# Autodesk Inventor assembly: Reactor Assembly
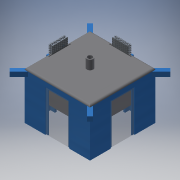
[picture p0: Inventor's stored thumbnail of the model, 180x180]
Saved by Autodesk Inventor 2017 (Build 210142000, 142)
## iProperties
Created: 2017-01-05
Part Number: Reactor Assembly
Document SubType Name: Assembly
Designer: jbui8
Author: jbui8
## Documents named in this file (5)
- C:\Users\jbui8\OneDrive\Documents\CAD Designs for Research and Work\PV Electrolyzer\Reactor Design\Reactor Parts\Assembly Parts\Reactor Assembly.iam
- C:\Users\jbui8\OneDrive\Documents\CAD Designs for Research and Work\PV Electrolyzer\Reactor Design\Reactor Parts\Assembly Parts\Reactor Main Body.ipt
- C:\Users\jbui8\OneDrive\Documents\CAD Designs for Research and Work\PV Electrolyzer\Reactor Design\Reactor Parts\Assembly Parts\Reactor Lid.ipt
- C:\Users\jbui8\OneDrive\Documents\CAD Designs for Research and Work\PV Electrolyzer\Reactor Design\Reactor Parts\Assembly Parts\Reactor Glass.ipt
- C:\Users\jbui8\OneDrive\Documents\CAD Designs for Research and Work\PV Electrolyzer\Reactor Design\Reactor Parts\Assembly Parts\Reactor Meshes.ipt
## Components (6 placed, 4 different names)
1. Reactor Main Body:1 — Mate:1, Mate:2, Mate:3, Mate:4, Mate:14, Mate:15, Mate:16, Mate:17, Mate:19, Mate:21
2. Reactor Lid:1 — Mate:2, Mate:3, Mate:4, Mate:18, Mate:20
3. Reactor Glass:1 — Mate:14, Mate:15
4. Reactor Glass:2 — Mate:16, Mate:17
5. Reactor Meshes:1 — Mate:18, Mate:19
6. Reactor Meshes:2 — Mate:20, Mate:21
## Relationships (12: Mate 12)
- Mate:1: Reactor Main Body:1
- Mate:2 (1 mm): Reactor Main Body:1 ↔ Reactor Lid:1
- Mate:3 (1 mm): Reactor Main Body:1 ↔ Reactor Lid:1
- Mate:4: Reactor Main Body:1 ↔ Reactor Lid:1
- Mate:14: Reactor Main Body:1 ↔ Reactor Glass:1
- Mate:15: Reactor Main Body:1 ↔ Reactor Glass:1
- Mate:16: Reactor Main Body:1 ↔ Reactor Glass:2
- Mate:17: Reactor Main Body:1 ↔ Reactor Glass:2
- Mate:18: Reactor Lid:1 ↔ Reactor Meshes:1
- Mate:19: Reactor Main Body:1 ↔ Reactor Meshes:1
- Mate:20: Reactor Lid:1 ↔ Reactor Meshes:2
- Mate:21: Reactor Main Body:1 ↔ Reactor Meshes:2
